# Autodesk Inventor assembly: Water system
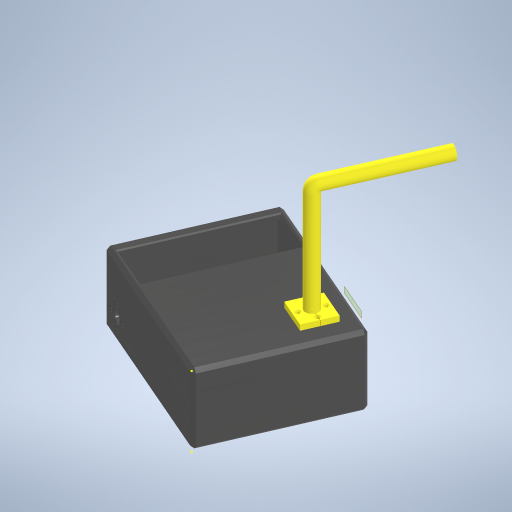
[picture p0: Inventor's stored thumbnail of the model, 512x512]
Saved by Autodesk Inventor 2023 (Build 270158000, 158)
## iProperties
Created: 2022-11-25
Part Number: Water system
Document SubType Name: Assembly
Designer: hp
Author: hp
## Documents named in this file (4)
- C:\Users\abdul\OneDrive\Skrivbord\maskin design\cad\ASS\System water kanjo.iam
- C:\Users\abdul\OneDrive\Skrivbord\maskin design\cad\ASS\Water container.ipt
- C:\Users\abdul\OneDrive\Skrivbord\maskin design\cad\ASS\water tube to pump.ipt
- C:\Users\abdul\OneDrive\Skrivbord\maskin design\cad\water to water container.ipt
## Components (3 placed, 3 different names)
1. Water container:1 — Mate:4, Mate:5, Mate:6, Mate:7, Mate:8
2. water tube to pump:1 — Mate:4, Mate:5
3. water to water container:1 — Mate:6, Mate:7, Mate:8
## Relationships (5: Mate 5)
- Mate:4: Water container:1 ↔ water tube to pump:1
- Mate:5: Water container:1 ↔ water tube to pump:1
- Mate:6: Water container:1 ↔ water to water container:1
- Mate:7: Water container:1 ↔ water to water container:1
- Mate:8: Water container:1 ↔ water to water container:1
